# Autodesk Inventor assembly: BREEZE-S08
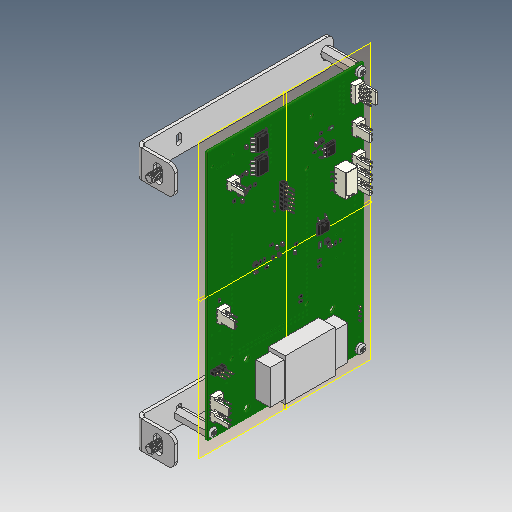
[picture p0: Inventor's stored thumbnail of the model, 512x512]
Saved by Autodesk Inventor 2020 (Build 240168000, 168)
## iProperties
Created: 2020-04-15
Part Number: BREEZE-S08
Document SubType Name: Assembly
Designer: John K
Description: PCB ASSEMBLY
Author: John K
## Documents named in this file (6)
- C:\GrabCAD\MTL Ventilator Design\BREEZE\Subassemblies\BREEZE-S08.iam
- C:\GrabCAD\MTL Ventilator Design\BREEZE\Manufactured Parts\PCB\PCB.iam
- C:\GrabCAD\MTL Ventilator Design\BREEZE\Manufactured Parts\BREEZE-M30.ipt
- C:\GrabCAD\MTL Ventilator Design\BREEZE\Commercial Parts\McMaster\M3 Standoff.ipt
- C:\GrabCAD\MTL Ventilator Design\BREEZE\Commercial Parts\McMaster\M3x6mm Nylon Screw.ipt
- C:\GrabCAD\MTL Ventilator Design\BREEZE\Commercial Parts\McMaster\M5x8mm Flanged Button.ipt
## Components (14 placed, 5 different names)
1. PCB:1 [sub-assembly] — Flush:1, Flush:2, Flush:3, Insert:1, Insert:2, Insert:3, Insert:5, Insert:6, Mate:12, Mate:13, Mate:14
2. BREEZE-M30:1 — Flush:4, Flush:5, Insert:7, Insert:8, Mate:5, Mate:6, Mate:7, Mate:11, Mate:12, Mate:13
3. BREEZE-M30:2 — Flush:4, Flush:5, Insert:9, Mate:8, Mate:10, Mate:14
4. M3 Standoff:1 — Insert:1, Insert:4, Mate:11
5. M3 Standoff:2 — Insert:2
6. M3 Standoff:3 — Insert:3
7. M3x6mm Nylon Screw:1 — Insert:4
8. M3x6mm Nylon Screw:2 — Insert:5
9. M3x6mm Nylon Screw:3 — Insert:6
10. M3x6mm Nylon Screw:4 — Insert:7
11. M3x6mm Nylon Screw:5 — Insert:8
12. M3x6mm Nylon Screw:6 — Insert:9
13. M5x8mm Flanged Button:1 — Mate:5, Mate:6, Mate:7, Mate:9
14. M5x8mm Flanged Button:2 — Mate:8, Mate:9, Mate:10
## Relationships (24: Mate 10, Insert 9, Flush 5)
- Flush:1: PCB:1
- Flush:2: PCB:1
- Flush:3: PCB:1
- Flush:4: BREEZE-M30:1 ↔ BREEZE-M30:2
- Flush:5: BREEZE-M30:1 ↔ BREEZE-M30:2
- Insert:1: PCB:1 ↔ M3 Standoff:1
- Insert:2: PCB:1 ↔ M3 Standoff:2
- Insert:3: PCB:1 ↔ M3 Standoff:3
- Insert:4: M3 Standoff:1 ↔ M3x6mm Nylon Screw:1
- Insert:5: PCB:1 ↔ M3x6mm Nylon Screw:2
- Insert:6: PCB:1 ↔ M3x6mm Nylon Screw:3
- Insert:7: BREEZE-M30:1 ↔ M3x6mm Nylon Screw:4
- Insert:8: BREEZE-M30:1 ↔ M3x6mm Nylon Screw:5
- Insert:9: BREEZE-M30:2 ↔ M3x6mm Nylon Screw:6
- Mate:5: BREEZE-M30:1 ↔ M5x8mm Flanged Button:1
- Mate:6 (2.7 mm): BREEZE-M30:1 ↔ M5x8mm Flanged Button:1
- Mate:7 (-9 mm): BREEZE-M30:1 ↔ M5x8mm Flanged Button:1
- Mate:8: BREEZE-M30:2 ↔ M5x8mm Flanged Button:2
- Mate:9: M5x8mm Flanged Button:1 ↔ M5x8mm Flanged Button:2
- Mate:10 (-9 mm): BREEZE-M30:2 ↔ M5x8mm Flanged Button:2
- Mate:11: BREEZE-M30:1 ↔ M3 Standoff:1
- Mate:12: PCB:1 ↔ BREEZE-M30:1
- Mate:13: PCB:1 ↔ BREEZE-M30:1
- Mate:14: PCB:1 ↔ BREEZE-M30:2
